# Autodesk Inventor assembly: MG-Kickerboard
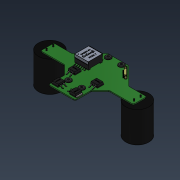
[picture p0: Inventor's stored thumbnail of the model, 180x180]
Saved by Autodesk Inventor 2022.1 (Build 261234020, 234B)
## iProperties
Part Number: MG-Kickerboard
Material: Generisch
Document SubType Name: Assembly
Designer: rYan
Mass: 155.116 g
Surface Area: 326.042 cm^2
Volume: 106.973 cm^3
Density: 1.45005 g/cm^3
Author: rYan
## Documents named in this file (7)
- D:\TIGERsGIT\Hardware\mechanik\2020\Inventor\Robot\Electronics\MG-Kickerboard.iam
- D:\TIGERsGIT\Hardware\mechanik\2020\Inventor\Robot\Electronics\Kickerboard.ipt
- D:\TIGERsGIT\Hardware\mechanik\2020\Inventor\Purchased Parts\Kondensator 30x40.ipt
- D:\TIGERsGIT\Hardware\mechanik\2020\Inventor\Purchased Parts\DF13C-12P-1.25V.ipt
- D:\TIGERsGIT\Hardware\mechanik\2020\Inventor\Purchased Parts\Gummitülle 3mm.ipt
- D:\TIGERsGIT\Hardware\mechanik\2020\Inventor\Purchased Parts\TO-263-3-2.ipt
- D:\TIGERsGIT\Hardware\mechanik\2020\Inventor\Purchased Parts\Coilcraft DA2034-AL.ipt
## Components (13 placed, 6 different names)
1. Kickerboard:1 — Einfügen:3, Einfügen:4, Passend:1, Passend:4, Passend:5, Passend:7, Einfügen:5, Einfügen:6, Einfügen:7, Einfügen:8, Passend:16, Fluchtend:3, Fluchtend:4, Passend:17, Fluchtend:5, Fluchtend:6, Passend:18, Passend:19, Fluchtend:9, Fluchtend:10, Fluchtend:11, Fluchtend:12, Fluchtend:13, Passend:20
2. Kondensator 30x40:1 — Einfügen:3, Passend:4
3. Kondensator 30x40:2 — Einfügen:4, Passend:1
4. DF13C-12P-1.25V:1 — Passend:5, Passend:7
5. Gummitülle 3mm:1 — Einfügen:5
6. Gummitülle 3mm:2 — Einfügen:6
7. Gummitülle 3mm:3 — Einfügen:7
8. Gummitülle 3mm:4 — Einfügen:8
9. TO-263-3-2:1 — Passend:17, Fluchtend:5, Fluchtend:6
10. TO-263-3-2:2 — Passend:16, Fluchtend:3, Fluchtend:4
11. TO-263-3-2:3 — Passend:18, Fluchtend:9, Fluchtend:10, Symmetrie:1, Symmetrie:2
12. TO-263-3-2:4 — Passend:19, Symmetrie:1, Symmetrie:2
13. Coilcraft DA2034-AL:1 — Passend:20, Fluchtend:14, Fluchtend:15
## Relationships (28: Flush 11, Mate 9, Insert 6, Symmetry 2)
- Einfügen:3 [Insert]: Kickerboard:1 ↔ Kondensator 30x40:1
- Einfügen:4 [Insert]: Kickerboard:1 ↔ Kondensator 30x40:2
- Passend:1 [Mate]: Kickerboard:1 ↔ Kondensator 30x40:2
- Passend:4 [Mate]: Kickerboard:1 ↔ Kondensator 30x40:1
- Passend:5 [Mate]: Kickerboard:1 ↔ DF13C-12P-1.25V:1
- Passend:7 [Mate] (-5 mm): Kickerboard:1 ↔ DF13C-12P-1.25V:1
- Einfügen:5 [Insert]: Kickerboard:1 ↔ Gummitülle 3mm:1
- Einfügen:6 [Insert]: Kickerboard:1 ↔ Gummitülle 3mm:2
- Einfügen:7 [Insert]: Kickerboard:1 ↔ Gummitülle 3mm:3
- Einfügen:8 [Insert]: Kickerboard:1 ↔ Gummitülle 3mm:4
- Passend:16 [Mate]: Kickerboard:1 ↔ TO-263-3-2:2
- Fluchtend:3 [Flush] (3 mm): Kickerboard:1 ↔ TO-263-3-2:2
- Fluchtend:4 [Flush] (1 mm): Kickerboard:1 ↔ TO-263-3-2:2
- Passend:17 [Mate]: Kickerboard:1 ↔ TO-263-3-2:1
- Fluchtend:5 [Flush] (3 mm): Kickerboard:1 ↔ TO-263-3-2:1
- Fluchtend:6 [Flush] (1 mm): Kickerboard:1 ↔ TO-263-3-2:1
- Passend:18 [Mate]: Kickerboard:1 ↔ TO-263-3-2:3
- Passend:19 [Mate]: Kickerboard:1 ↔ TO-263-3-2:4
- Fluchtend:9 [Flush] (-17 mm): Kickerboard:1 ↔ TO-263-3-2:3
- Fluchtend:10 [Flush] (-5 mm): Kickerboard:1 ↔ TO-263-3-2:3
- Symmetrie:1: TO-263-3-2:3 ↔ TO-263-3-2:4
- Symmetrie:2: TO-263-3-2:3 ↔ TO-263-3-2:4
- Fluchtend:11 [Flush]: Kickerboard:1
- Fluchtend:12 [Flush]: Kickerboard:1
- Fluchtend:13 [Flush]: Kickerboard:1
- Passend:20 [Mate]: Kickerboard:1 ↔ Coilcraft DA2034-AL:1
- Fluchtend:14 [Flush] (18.4 mm): Coilcraft DA2034-AL:1
- Fluchtend:15 [Flush] (-11.7 mm): Coilcraft DA2034-AL:1
